# Autodesk Inventor assembly: boot_mirror
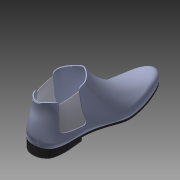
[picture p0: Inventor's stored thumbnail of the model, 180x180]
Saved by Autodesk Inventor 2016 (Build 200138000, 138)
## iProperties
Created: 2015-05-13
Part Number: boot_mirror
Document SubType Name: Assembly
Designer: Yann
Author: Yann
## Documents named in this file (3)
- C:\Users\Yann\Documents\GitHub\BIKAIR_CAD\Source\User\Source_SW\Accessories\boot_mirror.iam
- C:\Users\Yann\Documents\GitHub\BIKAIR_CAD\Source\User\Source_SW\Accessories\Boots.ipt
- C:\Users\Yann\Documents\GitHub\BIKAIR_CAD\Source\User\Source_SW\Accessories\Boots_MIR.ipt
## Components (2 placed, 2 different names)
1. Boots:1 — Flush:1, Flush:2, Flush:3
2. Boots_MIR:1 — Flush:4, Mate:1, Mate:2
## Relationships (6: Flush 4, Mate 2)
- Flush:1: Boots:1
- Flush:2: Boots:1
- Flush:3: Boots:1
- Flush:4: Boots_MIR:1
- Mate:1: Boots_MIR:1
- Mate:2: Boots_MIR:1
